# Autodesk Inventor assembly: spring
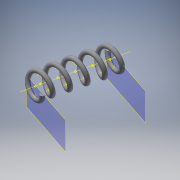
[picture p0: Inventor's stored thumbnail of the model, 180x180]
Saved by Autodesk Inventor 2017.2 (Build 212233000, 233)
## iProperties
Created: 2017-08-28
Part Number: spring
Document SubType Name: Assembly
Designer: Nic
Author: Nic
## Documents named in this file (2)
- C:\Users\Nic\Documents\iDripper\spring.iam
- C:\Users\Nic\Documents\iDripper\spring_part.ipt
## Components (11 placed, 1 different names)
1. spring_part:1 — Insert:2, Insert:3, Angle:8
2. spring_part:2 — Insert:3, Insert:4, Angle:2, Angle:3
3. spring_part:3 — Insert:1, Insert:2, Angle:2
4. spring_part:4 — Insert:1, Angle:13, Mate:2
5. spring_part:5 — Insert:4, Insert:5, Angle:8, Angle:12
6. spring_part:6 — Insert:5, Insert:6, Angle:3, Angle:4
7. spring_part:7 — Insert:9, Insert:10, Angle:5
8. spring_part:8 — Insert:8, Insert:9, Angle:9
9. spring_part:9 — Insert:7, Insert:8, Angle:4, Angle:5
10. spring_part:10 — Insert:10, Angle:13, Mate:1
11. spring_part:14 — Insert:6, Insert:7, Angle:9, Angle:12
## Relationships (20: Insert 10, Angle 8, Mate 2)
- Insert:1: spring_part:3 ↔ spring_part:4
- Insert:2: spring_part:1 ↔ spring_part:3
- Insert:3: spring_part:1 ↔ spring_part:2
- Insert:4: spring_part:2 ↔ spring_part:5
- Insert:5: spring_part:5 ↔ spring_part:6
- Insert:6: spring_part:6 ↔ spring_part:14
- Insert:7: spring_part:9 ↔ spring_part:14
- Insert:8: spring_part:8 ↔ spring_part:9
- Insert:9: spring_part:7 ↔ spring_part:8
- Insert:10: spring_part:7 ↔ spring_part:10
- Angle:2 (0 deg): spring_part:2 ↔ spring_part:3
- Angle:3 (0 deg): spring_part:2 ↔ spring_part:6
- Angle:4 (180 deg): spring_part:6 ↔ spring_part:9
- Angle:5 (0 deg): spring_part:7 ↔ spring_part:9
- Angle:8 (0 deg): spring_part:1 ↔ spring_part:5
- Angle:9 (0 deg): spring_part:8 ↔ spring_part:14
- Angle:12 (0 deg): spring_part:5 ↔ spring_part:14
- Angle:13 (0 deg): spring_part:4 ↔ spring_part:10
- Mate:1: spring_part:10
- Mate:2: spring_part:4
